# Autodesk Inventor assembly: CapLift2
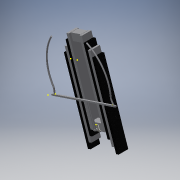
[picture p0: Inventor's stored thumbnail of the model, 180x180]
Saved by Autodesk Inventor 2017 (Build 210142000, 142)
## iProperties
Created: 2017-04-15
Part Number: CapLift2
Document SubType Name: Assembly
Designer: User
Author: User
## Documents named in this file (7)
- C:\Robotics\CAD\2016-17_CAD\CapLift2.iam
- C:\Robotics\CAD\2016-17_CAD\LiftSlidePart.ipt
- C:\Robotics\CAD\2016-17_CAD\Part2.ipt
- C:\Robotics\CAD\2016-17_CAD\slide pivot plate.0001 - Copy.ipt
- C:\Robotics\CAD\2016-17_CAD\HingeMK3Part3 - Copy.ipt
- C:\Robotics\CAD\2016-17_CAD\HingeMK3Part2 - Copy.ipt
- C:\Robotics\CAD\2016-17_CAD\CapBallHolderArmNew.ipt
## Components (15 placed, 6 different names)
1. LiftSlidePart:1 — Mate:7, Flush:11, Flush:12, Flush:13, Mate:9, Mate:10, Flush:17, Flush:18
2. LiftSlidePart:2 — Mate:5, Flush:7, Flush:8, Mate:6, Flush:9, Flush:10
3. LiftSlidePart:3 — Mate:5, Flush:7, Flush:8, Flush:14
4. LiftSlidePart:4 — Mate:6, Flush:9, Flush:10, Mate:7, Flush:11, Flush:12
5. LiftSlidePart:5 — Mate:4, Flush:5, Flush:6, Flush:13, Mate:8, Flush:15, Flush:16
6. LiftSlidePart:6 — Mate:2, Flush:1, Flush:2, Mate:3, Flush:3, Flush:4
7. LiftSlidePart:7 — Mate:2, Flush:1, Flush:2, Flush:14, Flush:20
8. LiftSlidePart:8 — Mate:3, Flush:3, Flush:4, Mate:4, Flush:5, Flush:6
9. Part2:1 — Mate:10, Flush:17, Flush:18, Mate:11, Flush:19
10. Part2:2 — Mate:8, Flush:15, Flush:16, Mate:9
11. slide pivot plate.0001 - Copy:1 — Mate:11, Flush:19, Flush:20, Mate:12, Mate:15, Flush:21
12. HingeMK3Part3 - Copy:1 — Mate:12, Mate:13, Mate:14
13. HingeMK3Part2 - Copy:1 — Mate:13, Mate:14, Mate:15, Flush:21, Mate:16, Mate:17
14. CapBallHolderArmNew:1 — Mate:16
15. CapBallHolderArmNew:2 — Mate:17
## Relationships (37: Flush 21, Mate 16)
- Mate:2: LiftSlidePart:6 ↔ LiftSlidePart:7
- Flush:1 (25.4 mm): LiftSlidePart:6 ↔ LiftSlidePart:7
- Flush:2: LiftSlidePart:6 ↔ LiftSlidePart:7
- Mate:3: LiftSlidePart:6 ↔ LiftSlidePart:8
- Flush:3 (25.4 mm): LiftSlidePart:6 ↔ LiftSlidePart:8
- Flush:4: LiftSlidePart:6 ↔ LiftSlidePart:8
- Mate:4: LiftSlidePart:5 ↔ LiftSlidePart:8
- Flush:5 (25.4 mm): LiftSlidePart:5 ↔ LiftSlidePart:8
- Flush:6: LiftSlidePart:5 ↔ LiftSlidePart:8
- Mate:5: LiftSlidePart:2 ↔ LiftSlidePart:3
- Flush:7 (25.4 mm): LiftSlidePart:2 ↔ LiftSlidePart:3
- Flush:8: LiftSlidePart:2 ↔ LiftSlidePart:3
- Mate:6: LiftSlidePart:2 ↔ LiftSlidePart:4
- Flush:9: LiftSlidePart:2 ↔ LiftSlidePart:4
- Flush:10 (25.4 mm): LiftSlidePart:2 ↔ LiftSlidePart:4
- Mate:7: LiftSlidePart:1 ↔ LiftSlidePart:4
- Flush:11 (25.4 mm): LiftSlidePart:1 ↔ LiftSlidePart:4
- Flush:12: LiftSlidePart:1 ↔ LiftSlidePart:4
- Flush:13: LiftSlidePart:1 ↔ LiftSlidePart:5
- Flush:14: LiftSlidePart:3 ↔ LiftSlidePart:7
- Mate:8: LiftSlidePart:5 ↔ Part2:2
- Flush:15: LiftSlidePart:5 ↔ Part2:2
- Flush:16 (8.255 mm): LiftSlidePart:5 ↔ Part2:2
- Mate:9: LiftSlidePart:1 ↔ Part2:2
- Mate:10: LiftSlidePart:1 ↔ Part2:1
- Flush:17: LiftSlidePart:1 ↔ Part2:1
- Flush:18: LiftSlidePart:1 ↔ Part2:1
- Mate:11: Part2:1 ↔ slide pivot plate.0001 - Copy:1
- Flush:19: Part2:1 ↔ slide pivot plate.0001 - Copy:1
- Flush:20 (59.69 mm): LiftSlidePart:7 ↔ slide pivot plate.0001 - Copy:1
- Mate:12: slide pivot plate.0001 - Copy:1 ↔ HingeMK3Part3 - Copy:1
- Mate:13: HingeMK3Part3 - Copy:1 ↔ HingeMK3Part2 - Copy:1
- Mate:14: HingeMK3Part3 - Copy:1 ↔ HingeMK3Part2 - Copy:1
- Mate:15 (0.508 mm): slide pivot plate.0001 - Copy:1 ↔ HingeMK3Part2 - Copy:1
- Flush:21: slide pivot plate.0001 - Copy:1 ↔ HingeMK3Part2 - Copy:1
- Mate:16: HingeMK3Part2 - Copy:1 ↔ CapBallHolderArmNew:1
- Mate:17: HingeMK3Part2 - Copy:1 ↔ CapBallHolderArmNew:2
